# Autodesk Inventor assembly: robotic arm
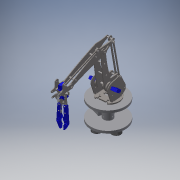
[picture p0: Inventor's stored thumbnail of the model, 180x180]
Saved by Autodesk Inventor 2017 SP1 (Build 210196100, 196)
## iProperties
Created: 2018-03-04
Part Number: robotic arm
Description: STEP AP214
Document SubType Name: Assembly
Designer: ANSHUL YADAV
Title: robotic arm.STEP
Revision Number: ANY
Sending System: SolidWorks 2018
Preprocessor: SwSTEP 2.0
## Documents named in this file (25)
- H:\Robotics@IITD\robotic arm.iam
- H:\Robotics@IITD\Part13.ipt
- H:\Robotics@IITD\parallel pin hardened_iso_ISO 8734 - 8 x 50 - A - St.ipt
- H:\Robotics@IITD\spring pin slotted_ld_iso_ISO 13337 - 5 x 28 - St.ipt
- H:\Robotics@IITD\Part 9.ipt
- H:\Robotics@IITD\Servo Motor Assembly.iam
- H:\Robotics@IITD\Part1^Assem4 lay out.ipt
- H:\Robotics@IITD\Part2^Assem4.ipt
- H:\Robotics@IITD\Part1^Assem4.ipt
- H:\Robotics@IITD\Part1^Assem4_1.ipt
- H:\Robotics@IITD\washer.ipt
- H:\Robotics@IITD\Part6^Assem4.ipt
- H:\Robotics@IITD\Part4^Assem4.ipt
- H:\Robotics@IITD\Part3^Assem4.ipt
- H:\Robotics@IITD\Part5^Assem4.ipt
- H:\Robotics@IITD\Part7^Assem4.ipt
- H:\Robotics@IITD\spring pin slotted_ld_iso_ISO 13337 - 6 x 22 - St.ipt
- H:\Robotics@IITD\pan head cross recess screw_iso_ISO 7045 - M3 x 30 - Z - 30S.ipt
- H:\Robotics@IITD\hex thin nut chamfered gradeab_iso_ISO - 4035 - M3 - S.ipt
- H:\Robotics@IITD\plain washer 10669 type nl_iso_ISO 10669-4.7-N.ipt
- H:\Robotics@IITD\pan head cross recess screw_iso_ISO 7045 - M4 x 12 - Z - 12S.ipt
- H:\Robotics@IITD\pan head cross recess screw_iso_ISO 7045 - M4 x 8 - Z - 8S.ipt
- H:\Robotics@IITD\hex thin nut chamfered gradeab_iso_ISO - 4035 - M4 - S.ipt
- H:\Robotics@IITD\Gripper assem.iam
- H:\Robotics@IITD\My Assebly\Turntable.iam
## Components (52 placed, 52 different names)
1. Part13_3 — Mate:3, Mate:12
2. Part13_4 — Mate:4, Mate:10
3. Part13_5 — Mate:2, Mate:11
4. parallel pin hardened_iso_ISO 8734 - 8 x 50 - A - St_23
5. spring pin slotted_ld_iso_ISO 13337 - 5 x 28 - St_24
6. spring pin slotted_ld_iso_ISO 13337 - 5 x 28 - St_25
7. Part 9_27 — Mate:5, Mate:6, Mate:7, Mate:8, Mate:9
8. Servo Motor Assembly_29 [sub-assembly]
9. Servo Motor Assembly_30 [sub-assembly]
10. Part1^Assem4 lay out_31 — Mate:5, Mate:7
11. Part1^Assem4 lay out_32 — Mate:6, Mate:8
12. Part2^Assem4_33
13. Part1^Assem4_34
14. Part1^Assem4_35
15. washer_36
16. Part6^Assem4_37
17. Part4^Assem4_38
18. Part4^Assem4_39
19. Part3^Assem4_40
20. Part5^Assem4_41
21. Part7^Assem4_42
22. washer_43
23. Part7^Assem4_44
24. spring pin slotted_ld_iso_ISO 13337 - 6 x 22 - St_45
25. spring pin slotted_ld_iso_ISO 13337 - 6 x 22 - St_46
26. spring pin slotted_ld_iso_ISO 13337 - 6 x 22 - St_47
27. spring pin slotted_ld_iso_ISO 13337 - 6 x 22 - St_48
28. spring pin slotted_ld_iso_ISO 13337 - 6 x 22 - St_49
29. pan head cross recess screw_iso_ISO 7045 - M3 x 30 - Z - 30S_50
30. pan head cross recess screw_iso_ISO 7045 - M3 x 30 - Z - 30S_51
31. pan head cross recess screw_iso_ISO 7045 - M3 x 30 - Z - 30S_52
32. pan head cross recess screw_iso_ISO 7045 - M3 x 30 - Z - 30S_53
33. hex thin nut chamfered gradeab_iso_ISO - 4035 - M3 - S_54
34. hex thin nut chamfered gradeab_iso_ISO - 4035 - M3 - S_55
35. hex thin nut chamfered gradeab_iso_ISO - 4035 - M3 - S_56
36. hex thin nut chamfered gradeab_iso_ISO - 4035 - M3 - S_57
37. hex thin nut chamfered gradeab_iso_ISO - 4035 - M3 - S_58
38. hex thin nut chamfered gradeab_iso_ISO - 4035 - M3 - S_59
39. plain washer 10669 type nl_iso_ISO 10669-4.7-N_60
40. pan head cross recess screw_iso_ISO 7045 - M4 x 12 - Z - 12S_61
41. pan head cross recess screw_iso_ISO 7045 - M4 x 8 - Z - 8S_62
42. hex thin nut chamfered gradeab_iso_ISO - 4035 - M4 - S_63
43. hex thin nut chamfered gradeab_iso_ISO - 4035 - M4 - S_64
44. pan head cross recess screw_iso_ISO 7045 - M4 x 8 - Z - 8S_65
45. hex thin nut chamfered gradeab_iso_ISO - 4035 - M4 - S_66
46. pan head cross recess screw_iso_ISO 7045 - M3 x 30 - Z - 30S_67
47. pan head cross recess screw_iso_ISO 7045 - M3 x 30 - Z - 30S_68
48. pan head cross recess screw_iso_ISO 7045 - M3 x 30 - Z - 30S_69
49. hex thin nut chamfered gradeab_iso_ISO - 4035 - M4 - S_70
50. Gripper assem_71 [sub-assembly]
51. Turntable:1 [sub-assembly] — Mate:2, Mate:3, Mate:4, Mate:9, Mate:10, Mate:11, Mate:12, Mate:13
52. Part13:5 — Mate:13
## Relationships (12: Mate 12)
- Mate:2: Part13_5 ↔ Turntable:1
- Mate:3: Part13_3 ↔ Turntable:1
- Mate:4: Part13_4 ↔ Turntable:1
- Mate:5: Part 9_27 ↔ Part1^Assem4 lay out_31
- Mate:6: Part 9_27 ↔ Part1^Assem4 lay out_32
- Mate:7: Part 9_27 ↔ Part1^Assem4 lay out_31
- Mate:8: Part 9_27 ↔ Part1^Assem4 lay out_32
- Mate:9: Part 9_27 ↔ Turntable:1
- Mate:10: Part13_4 ↔ Turntable:1
- Mate:11: Part13_5 ↔ Turntable:1
- Mate:12: Part13_3 ↔ Turntable:1
- Mate:13: Turntable:1 ↔ Part13:5
